# Autodesk Inventor assembly: T04
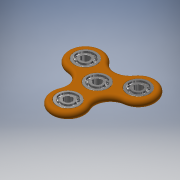
[picture p0: Inventor's stored thumbnail of the model, 180x180]
Saved by Autodesk Inventor 2018 (Build 220112000, 112)
## iProperties
Created: 2020-06-26
Part Number: T04
Document SubType Name: Assembly
Designer: BLACK_HOLE
Author: BLACK_HOLE
## Documents named in this file (4)
- F:\Users\Desktop\Desktop\Clase de Proyectos\Modelos Inventor\Spinner\T04_Max\T04.iam
- F:\Users\Desktop\Desktop\Clase de Proyectos\Modelos Inventor\Spinner\principal.ipt
- F:\Users\Desktop\Desktop\Clase de Proyectos\Modelos Inventor\Spinner\Assembly1\Design Accelerator\Bearing1.iam
- F:\Users\Desktop\Desktop\Clase de Proyectos\Modelos Inventor\Spinner\Assembly1\Design Accelerator\Bearing2.iam
## Components (5 placed, 2 different names)
1. principal:1 — Mate:1, Mate:2, Mate:3, Mate:4, Mate:5
2. Bearing:1 [sub-assembly] — Mate:1, Mate:2, Mate:5, Mate:6
3. Bearing:2 [sub-assembly] — Mate:3, Mate:4
4. Bearing:3 [sub-assembly]
5. Bearing:4 [sub-assembly]
## Component patterns: (3 elements, first: Bearing:2)
## Relationships (6: Mate 6)
- Mate:1: principal:1 ↔ Bearing:1
- Mate:2: principal:1 ↔ Bearing:1
- Mate:3: principal:1 ↔ Bearing:2
- Mate:4: principal:1 ↔ Bearing:2
- Mate:5: principal:1 ↔ Bearing:1
- Mate:6: Bearing:1
